# Autodesk Inventor assembly: NEMA_14HM11-0404S
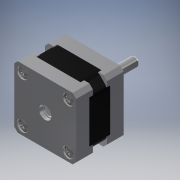
[picture p0: Inventor's stored thumbnail of the model, 180x180]
Saved by Autodesk Inventor 2019.4 (Build 234330000, 330)
## iProperties
Created: 2019-11-25
Part Number: NEMA_14HM11-0404S
Material: Générique
Document SubType Name: Assembly
Designer: thoma
Author: thoma
## Documents named in this file (4)
- C:\Users\thoma\Documents\GrabCAD\smart-bowl\actuators\NEMA_14HM11-0404S.iam
- C:\Users\thoma\Documents\GrabCAD\smart-bowl\actuators\NEMA_14HM11-0404S_BODY.ipt
- C:\Users\thoma\Documents\GrabCAD\smart-bowl\actuators\NEMA_14HM11-0404S_SHAFT.ipt
- C:\Users\thoma\Documents\Inventor\Content Center Files\R2019\fr-FR\JIS B 1111 (H) (2)\JIS B 1111 (H) - M3x6 - 4.8(2).ipt
## Components (6 placed, 3 different names)
1. NEMA_14HM11-0404S:1 — Affleurement:2, Placage:2, Placage:3, Affleurement:3, Placage:4, Rigide:1
2. NEMA_14HM11-0404S_SHAFT:1 — Affleurement:3
3. JIS B 1111 (H) M3x6 - 4.8:1 — Placage:4
4. JIS B 1111 (H) M3x6 - 4.8:2 — Rigide:1
5. JIS B 1111 (H) M3x6 - 4.8:3
6. JIS B 1111 (H) M3x6 - 4.8:4
## Component patterns: (4 elements, first: JIS B 1111 (H) M3x6 - 4.8:1)
## Relationships (6: Mate 3, Flush 2, WeldJoint 1)
- Affleurement:2 [Flush]: NEMA_14HM11-0404S:1
- Placage:2 [Mate]: NEMA_14HM11-0404S:1
- Placage:3 [Mate]: NEMA_14HM11-0404S:1
- Affleurement:3 [Flush]: NEMA_14HM11-0404S:1 ↔ NEMA_14HM11-0404S_SHAFT:1
- Placage:4 [Mate]: NEMA_14HM11-0404S:1 ↔ JIS B 1111 (H) M3x6 - 4.8:1
- Rigide:1 [WeldJoint] (1.5 mm): NEMA_14HM11-0404S:1 ↔ JIS B 1111 (H) M3x6 - 4.8:2
